# Autodesk Inventor assembly: UBG-Kamera mit Halter geneigt
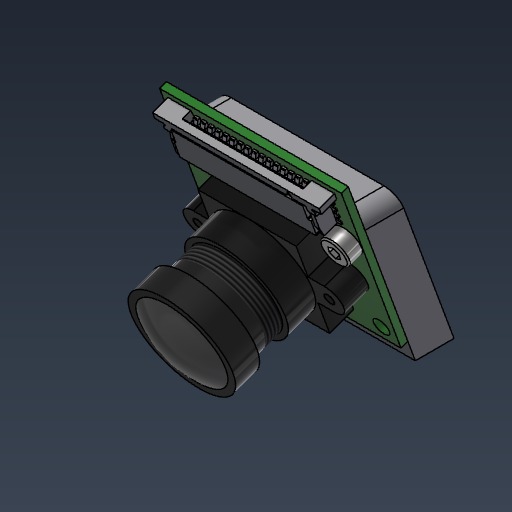
[picture p0: Inventor's stored thumbnail of the model, 512x512]
Saved by Autodesk Inventor 2023.1 (Build 271208000, 208)
## iProperties
Part Number: UBG-Kamera mit Halter geneigt
Material: Generisch
Document SubType Name: Assembly
Designer: rYan
Mass: 4.8103 g
Surface Area: 57.9184 cm^2
Volume: 5.00584 cm^3
Density: 0.960938 g/cm^3
Author: rYan
## Documents named in this file (4)
- D:\TIGERsGIT\Hardware\mechanik\2024\Inventor\Robot\Electronics\UBG-Kamera mit Halter geneigt.iam
- D:\TIGERsGIT\Hardware\mechanik\2024\Inventor\Robot\Electronics\Kamerahalter Vorne geneigt.ipt
- D:\TIGERsGIT\Hardware\mechanik\2024\Inventor\Purchased Parts\Waveshare Kamera 25x24\MG-Waveshare Kamera 25x24.iam
- D:\TIGERsGIT\Hardware\mechanik\2024\Inventor\Inhaltscenter\de-DE\ISO 4762(2)\ISO 4762 - M2 x 6ISO.ipt
## Components (4 placed, 3 different names)
1. Kamerahalter Vorne geneigt:1 — Einfügen:1, Einfügen:2
2. MG-Waveshare Kamera 25x24:1 [sub-assembly] — Einfügen:1, Einfügen:2, Einfügen:3, Einfügen:4
3. ISO 4762 M2 x 6:1 — Einfügen:3
4. ISO 4762 M2 x 6:2 — Einfügen:4
## Relationships (4: Insert 4)
- Einfügen:1 [Insert]: Kamerahalter Vorne geneigt:1 ↔ MG-Waveshare Kamera 25x24:1
- Einfügen:2 [Insert]: Kamerahalter Vorne geneigt:1 ↔ MG-Waveshare Kamera 25x24:1
- Einfügen:3 [Insert]: MG-Waveshare Kamera 25x24:1 ↔ ISO 4762 M2 x 6:1
- Einfügen:4 [Insert]: MG-Waveshare Kamera 25x24:1 ↔ ISO 4762 M2 x 6:2
